# Autodesk Inventor assembly: Manipulator
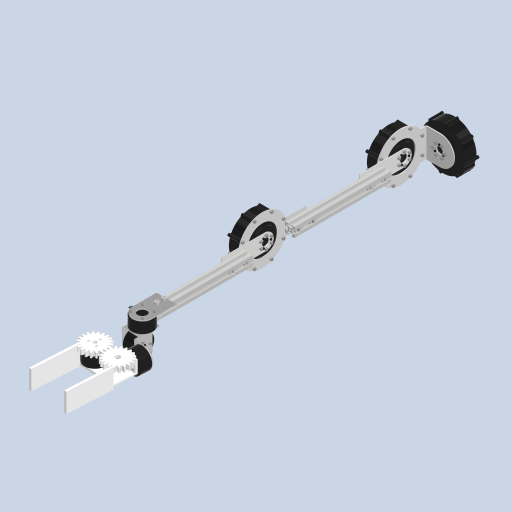
[picture p0: Inventor's stored thumbnail of the model, 512x512]
Saved by Autodesk Inventor 2023 (Build 270158000, 158)
## iProperties
Created: 2024-11-08
Part Number: Manipulator
Document SubType Name: Assembly
Designer: kiyo
Author: kiyo
## Documents named in this file (20)
- D:\GitHub\inventor\syu-si\OfficeRobot\Manipulator\Manipulator.iam
- D:\GitHub\inventor\syu-si\OfficeRobot\ReadyMade\Steadywin\GIM8108-8.iam
- D:\GitHub\inventor\syu-si\OfficeRobot\Manipulator\sholder-roll-bracket.ipt
- D:\GitHub\inventor\syu-si\OfficeRobot\Manipulator\shoulder_pitch_plate.ipt
- D:\GitHub\inventor\syu-si\OfficeRobot\Manipulator\elbow-pitch-bracket.ipt
- D:\GitHub\inventor\syu-si\OfficeRobot\Manipulator\Hand.iam
- D:\GitHub\inventor\syu-si\OfficeRobot\Manipulator\wrist-pitch-plate.ipt
- D:\GitHub\inventor\syu-si\OfficeRobot\Manipulator\wrist-yaw-plate.ipt
- D:\GitHub\inventor\syu-si\OfficeRobot\ReadyMade\Steadywin\GIM3505-8.ipt
- D:\GitHub\inventor\syu-si\OfficeRobot\Manipulator\wrist_roll_plate.ipt
- D:\GitHub\inventor\syu-si\OfficeRobot\Manipulator\HFS5-2020-200-Z5-XA10-XB40-XC160-XD190.ipt
- D:\GitHub\inventor\syu-si\OfficeRobot\ReadyMade\Screw\M3_7mm.ipt
- D:\GitHub\inventor\syu-si\OfficeRobot\ReadyMade\Screw\M3_6mm.ipt
- D:\GitHub\inventor\syu-si\OfficeRobot\ReadyMade\Screw\M2-5_4mm.ipt
- D:\GitHub\inventor\syu-si\OfficeRobot\ReadyMade\Screw\M2-5_5mm.ipt
- D:\GitHub\inventor\syu-si\OfficeRobot\ReadyMade\Screw\M2-5_7mm.ipt
- D:\GitHub\inventor\syu-si\OfficeRobot\ReadyMade\Screw\SCB5-22.ipt
- D:\GitHub\inventor\syu-si\OfficeRobot\ReadyMade\Screw\HNTP5-5.ipt
- D:\GitHub\inventor\syu-si\OfficeRobot\ReadyMade\Screw\HNTT5-5.ipt
- D:\GitHub\inventor\syu-si\OfficeRobot\ReadyMade\Screw\SCB5-8.ipt
## Components (95 placed, 19 different names)
1. GIM8108-8:1 [sub-assembly] — 挿入:1
2. GIM8108-8:2 [sub-assembly] — 挿入:2, 挿入:3, 挿入:4
3. GIM8108-8:3 [sub-assembly] — 挿入:7, 挿入:21, 挿入:22
4. sholder-roll-bracket:1 — 挿入:1, 挿入:2, 挿入:3, 肩ヨー, 挿入:94, 挿入:95, 挿入:96, 挿入:97, 挿入:98, 挿入:99, 挿入:100, 挿入:101, 挿入:102, 挿入:103, 挿入:104, 挿入:105, 挿入:106, 挿入:107
5. shoulder_pitch_plate:1 — 挿入:4, 肩ピッチ, 挿入:17, 挿入:18, 挿入:108, 挿入:109, 挿入:110, 挿入:111, 挿入:112, 挿入:113, 挿入:151, 挿入:152
6. elbow-pitch-bracket:1 — 挿入:19, 挿入:20, 挿入:21, 挿入:22, 挿入:86, 挿入:87, 挿入:88, 挿入:89, 挿入:90, 挿入:91, 挿入:92, 挿入:93, 挿入:153, 挿入:154
7. shoulder_pitch_plate:2 — 挿入:7, 肘ピッチ, 挿入:23, 挿入:24, 挿入:114, 挿入:115, 挿入:116, 挿入:117, 挿入:118, 挿入:119, 挿入:149, 挿入:150
8. GIM3505-8:1 — 挿入:63, 挿入:64, 挿入:79
9. GIM3505-8:2 — 挿入:13, 挿入:80, 挿入:81
10. GIM3505-8:3 — 挿入:16, 挿入:57, 挿入:58
11. wrist-yaw-plate:1 — メイト:1, メイト:2, フラッシュ:1, 挿入:63, 挿入:64, 挿入:120, 挿入:121, 挿入:122, 挿入:123, 挿入:161, 挿入:162, 挿入:163, 挿入:164
12. wrist_roll_plate:1 — 挿入:13, 手首ピッチ, 挿入:57, 挿入:58, 挿入:135, 挿入:136, 挿入:137, 挿入:145, 挿入:146, 挿入:147, 挿入:148
13. wrist-pitch-plate:1 — 挿入:79, 挿入:80, 挿入:81, 挿入:124, 挿入:125, 挿入:126, 挿入:127, 挿入:132, 挿入:133, 挿入:134
14. HFS5-2020-200-Z5-XA10-XB40-XC160-XD190:1 — 挿入:17, 挿入:18, 挿入:19, 挿入:20, 挿入:155, 挿入:156, 挿入:159, 挿入:160, 角度:11, 角度:12, 角度:13, 角度:14
15. HFS5-2020-200-Z5-XA10-XB40-XC160-XD190:2 — 挿入:23, 挿入:24, メイト:1, メイト:2, フラッシュ:1, 挿入:157, 挿入:158, 角度:7, 角度:8, 角度:9, 角度:10
16. Hand:1 [sub-assembly] — 挿入:16, ハンド, 挿入:128, 挿入:129, 挿入:130, 挿入:131, 挿入:138, 挿入:139, 挿入:140, 挿入:141, 挿入:142, 挿入:143, 挿入:144
17. M3_6mm:1 — 挿入:108
18. M3_6mm:2 — 挿入:110
19. M3_6mm:3 — 挿入:111
20. M3_6mm:4 — 挿入:112
21. M3_6mm:5 — 挿入:113
22. M3_6mm:6 — 挿入:109
23. M3_6mm:7 — 挿入:118
24. M3_6mm:8 — 挿入:117
25. M3_6mm:9 — 挿入:116
26. M3_6mm:10 — 挿入:115
27. M3_6mm:11 — 挿入:114
28. M3_6mm:12 — 挿入:119
29. M3_6mm:13 — 挿入:107
30. M3_6mm:14 — 挿入:106
31. M3_6mm:15 — 挿入:105
32. M3_6mm:16 — 挿入:102
33. M3_6mm:17 — 挿入:103
34. M3_6mm:18 — 挿入:104
35. M3_7mm:1 — 挿入:144
36. M3_7mm:2 — 挿入:101
37. M3_7mm:3 — 挿入:100
38. M3_7mm:4 — 挿入:99
39. M3_7mm:5 — 挿入:97
40. M3_7mm:6 — 挿入:98
41. M3_7mm:7 — 挿入:96
42. M3_7mm:8 — 挿入:95
43. M3_7mm:9 — 挿入:94
44. M3_7mm:10 — 挿入:92
45. M3_7mm:11 — 挿入:93
46. M3_7mm:12 — 挿入:86
47. M3_7mm:13 — 挿入:87
48. M3_7mm:14 — 挿入:91
49. M3_7mm:15 — 挿入:90
50. M3_7mm:16 — 挿入:89
51. M3_7mm:17 — 挿入:88
52. M2-5_4mm:21 — 挿入:147
53. M2-5_4mm:22 — 挿入:146
54. M2-5_4mm:23 — 挿入:145
55. M2-5_4mm:24 — 挿入:148
56. M2-5_4mm:1 — 挿入:120
57. M2-5_4mm:2 — 挿入:126
58. M2-5_4mm:3 — 挿入:125
59. M2-5_4mm:4 — 挿入:122
60. M2-5_4mm:5 — 挿入:121
61. M2-5_4mm:6 — 挿入:127
62. M2-5_4mm:7 — 挿入:124
63. M2-5_4mm:8 — 挿入:123
64. M2-5_4mm:9 — 挿入:129
65. M2-5_4mm:10 — 挿入:130
66. M2-5_4mm:11 — 挿入:131
67. M2-5_4mm:12 — 挿入:128
68. M2-5_5mm:1 — 挿入:132
69. M2-5_5mm:2 — 挿入:134
70. M2-5_5mm:3 — 挿入:133
71. M2-5_5mm:4 — 挿入:135
72. M2-5_5mm:5 — 挿入:137
73. M2-5_5mm:6 — 挿入:136
74. M2-5_5mm:7 — 挿入:138
75. M2-5_5mm:8 — 挿入:139
76. M2-5_5mm:9 — 挿入:140
77. M2-5_7mm:1 — 挿入:141
78. M2-5_7mm:2 — 挿入:142
79. M2-5_7mm:3 — 挿入:143
80. SCB5-22:1 — 挿入:153
81. SCB5-22:2 — 挿入:154
82. SCB5-22:3 — 挿入:152
83. SCB5-22:4 — 挿入:151
84. SCB5-22:5 — 挿入:150
85. SCB5-22:6 — 挿入:149
86. HNTP5-5:1 — 挿入:158, 角度:10
87. HNTP5-5:2 — 挿入:157, 角度:9
88. HNTP5-5:3 — 挿入:156, 角度:12
89. HNTP5-5:4 — 挿入:155, 角度:11
90. HNTP5-5:7 — 挿入:159, 角度:13
91. HNTP5-5:8 — 挿入:160, 角度:14
92. HNTT5-5:1 — 挿入:161, 角度:7
93. HNTT5-5:2 — 挿入:162, 角度:8
94. SCB5-8:1 — 挿入:163
95. SCB5-8:2 — 挿入:164
## Relationships (117: Insert 101, Angle 13, Mate 2, Flush 1)
- 挿入:1 [Insert]: GIM8108-8:1 ↔ sholder-roll-bracket:1
- 挿入:2 [Insert]: GIM8108-8:2 ↔ sholder-roll-bracket:1
- 挿入:3 [Insert]: GIM8108-8:2 ↔ sholder-roll-bracket:1
- 挿入:4 [Insert]: GIM8108-8:2 ↔ shoulder_pitch_plate:1
- 挿入:7 [Insert]: GIM8108-8:3 ↔ shoulder_pitch_plate:2
- 挿入:13 [Insert]: GIM3505-8:2 ↔ wrist_roll_plate:1
- 挿入:16 [Insert]: GIM3505-8:3 ↔ Hand:1
- 肩ヨー [Angle] (0 deg): sholder-roll-bracket:1
- 肩ピッチ [Angle] (0 deg): shoulder_pitch_plate:1
- 肘ピッチ [Angle] (0 deg): shoulder_pitch_plate:2
- 手首ピッチ [Angle] (0 deg): wrist_roll_plate:1
- ハンド [Angle] (0 deg): Hand:1
- 挿入:17 [Insert] (6 mm): shoulder_pitch_plate:1 ↔ HFS5-2020-200-Z5-XA10-XB40-XC160-XD190:1
- 挿入:18 [Insert] (6 mm): shoulder_pitch_plate:1 ↔ HFS5-2020-200-Z5-XA10-XB40-XC160-XD190:1
- 挿入:19 [Insert] (6 mm): elbow-pitch-bracket:1 ↔ HFS5-2020-200-Z5-XA10-XB40-XC160-XD190:1
- 挿入:20 [Insert] (6 mm): elbow-pitch-bracket:1 ↔ HFS5-2020-200-Z5-XA10-XB40-XC160-XD190:1
- 挿入:21 [Insert]: GIM8108-8:3 ↔ elbow-pitch-bracket:1
- 挿入:22 [Insert]: GIM8108-8:3 ↔ elbow-pitch-bracket:1
- 挿入:23 [Insert] (6 mm): shoulder_pitch_plate:2 ↔ HFS5-2020-200-Z5-XA10-XB40-XC160-XD190:2
- 挿入:24 [Insert] (6 mm): shoulder_pitch_plate:2 ↔ HFS5-2020-200-Z5-XA10-XB40-XC160-XD190:2
- メイト:1 [Mate] (-30 mm): wrist-yaw-plate:1 ↔ HFS5-2020-200-Z5-XA10-XB40-XC160-XD190:2
- メイト:2 [Mate]: wrist-yaw-plate:1 ↔ HFS5-2020-200-Z5-XA10-XB40-XC160-XD190:2
- フラッシュ:1 [Flush] (-10.5 mm): wrist-yaw-plate:1 ↔ HFS5-2020-200-Z5-XA10-XB40-XC160-XD190:2
- 挿入:57 [Insert]: GIM3505-8:3 ↔ wrist_roll_plate:1
- 挿入:58 [Insert]: GIM3505-8:3 ↔ wrist_roll_plate:1
- 挿入:63 [Insert]: GIM3505-8:1 ↔ wrist-yaw-plate:1
- 挿入:64 [Insert]: GIM3505-8:1 ↔ wrist-yaw-plate:1
- 挿入:79 [Insert]: GIM3505-8:1 ↔ wrist-pitch-plate:1
- 挿入:80 [Insert]: GIM3505-8:2 ↔ wrist-pitch-plate:1
- 挿入:81 [Insert]: GIM3505-8:2 ↔ wrist-pitch-plate:1
- 挿入:86 [Insert]: elbow-pitch-bracket:1 ↔ M3_7mm:12
- 挿入:87 [Insert]: elbow-pitch-bracket:1 ↔ M3_7mm:13
- 挿入:88 [Insert]: elbow-pitch-bracket:1 ↔ M3_7mm:17
- 挿入:89 [Insert]: elbow-pitch-bracket:1 ↔ M3_7mm:16
- 挿入:90 [Insert]: elbow-pitch-bracket:1 ↔ M3_7mm:15
- 挿入:91 [Insert]: elbow-pitch-bracket:1 ↔ M3_7mm:14
- 挿入:92 [Insert]: elbow-pitch-bracket:1 ↔ M3_7mm:10
- 挿入:93 [Insert]: elbow-pitch-bracket:1 ↔ M3_7mm:11
- 挿入:94 [Insert]: sholder-roll-bracket:1 ↔ M3_7mm:9
- 挿入:95 [Insert]: sholder-roll-bracket:1 ↔ M3_7mm:8
- 挿入:96 [Insert]: sholder-roll-bracket:1 ↔ M3_7mm:7
- 挿入:97 [Insert]: sholder-roll-bracket:1 ↔ M3_7mm:5
- 挿入:98 [Insert]: sholder-roll-bracket:1 ↔ M3_7mm:6
- 挿入:99 [Insert]: sholder-roll-bracket:1 ↔ M3_7mm:4
- 挿入:100 [Insert]: sholder-roll-bracket:1 ↔ M3_7mm:3
- 挿入:101 [Insert]: sholder-roll-bracket:1 ↔ M3_7mm:2
- 挿入:102 [Insert]: sholder-roll-bracket:1 ↔ M3_6mm:16
- 挿入:103 [Insert]: sholder-roll-bracket:1 ↔ M3_6mm:17
- 挿入:104 [Insert]: sholder-roll-bracket:1 ↔ M3_6mm:18
- 挿入:105 [Insert]: sholder-roll-bracket:1 ↔ M3_6mm:15
- 挿入:106 [Insert]: sholder-roll-bracket:1 ↔ M3_6mm:14
- 挿入:107 [Insert]: sholder-roll-bracket:1 ↔ M3_6mm:13
- 挿入:108 [Insert]: shoulder_pitch_plate:1 ↔ M3_6mm:1
- 挿入:109 [Insert]: shoulder_pitch_plate:1 ↔ M3_6mm:6
- 挿入:110 [Insert]: shoulder_pitch_plate:1 ↔ M3_6mm:2
- 挿入:111 [Insert]: shoulder_pitch_plate:1 ↔ M3_6mm:3
- 挿入:112 [Insert]: shoulder_pitch_plate:1 ↔ M3_6mm:4
- 挿入:113 [Insert]: shoulder_pitch_plate:1 ↔ M3_6mm:5
- 挿入:114 [Insert]: shoulder_pitch_plate:2 ↔ M3_6mm:11
- 挿入:115 [Insert]: shoulder_pitch_plate:2 ↔ M3_6mm:10
- 挿入:116 [Insert]: shoulder_pitch_plate:2 ↔ M3_6mm:9
- 挿入:117 [Insert]: shoulder_pitch_plate:2 ↔ M3_6mm:8
- 挿入:118 [Insert]: shoulder_pitch_plate:2 ↔ M3_6mm:7
- 挿入:119 [Insert]: shoulder_pitch_plate:2 ↔ M3_6mm:12
- 挿入:120 [Insert]: wrist-yaw-plate:1 ↔ M2-5_4mm:1
- 挿入:121 [Insert]: wrist-yaw-plate:1 ↔ M2-5_4mm:5
- 挿入:122 [Insert]: wrist-yaw-plate:1 ↔ M2-5_4mm:4
- 挿入:123 [Insert]: wrist-yaw-plate:1 ↔ M2-5_4mm:8
- 挿入:124 [Insert]: wrist-pitch-plate:1 ↔ M2-5_4mm:7
- 挿入:125 [Insert]: wrist-pitch-plate:1 ↔ M2-5_4mm:3
- 挿入:126 [Insert]: wrist-pitch-plate:1 ↔ M2-5_4mm:2
- 挿入:127 [Insert]: wrist-pitch-plate:1 ↔ M2-5_4mm:6
- 挿入:128 [Insert]: Hand:1 ↔ M2-5_4mm:12
- 挿入:129 [Insert]: Hand:1 ↔ M2-5_4mm:9
- 挿入:130 [Insert]: Hand:1 ↔ M2-5_4mm:10
- 挿入:131 [Insert]: Hand:1 ↔ M2-5_4mm:11
- 挿入:132 [Insert]: wrist-pitch-plate:1 ↔ M2-5_5mm:1
- 挿入:133 [Insert]: wrist-pitch-plate:1 ↔ M2-5_5mm:3
- 挿入:134 [Insert]: wrist-pitch-plate:1 ↔ M2-5_5mm:2
- 挿入:135 [Insert]: wrist_roll_plate:1 ↔ M2-5_5mm:4
- 挿入:136 [Insert]: wrist_roll_plate:1 ↔ M2-5_5mm:6
- 挿入:137 [Insert]: wrist_roll_plate:1 ↔ M2-5_5mm:5
- 挿入:138 [Insert]: Hand:1 ↔ M2-5_5mm:7
- 挿入:139 [Insert]: Hand:1 ↔ M2-5_5mm:8
- 挿入:140 [Insert]: Hand:1 ↔ M2-5_5mm:9
- 挿入:141 [Insert]: Hand:1 ↔ M2-5_7mm:1
- 挿入:142 [Insert]: Hand:1 ↔ M2-5_7mm:2
- 挿入:143 [Insert]: Hand:1 ↔ M2-5_7mm:3
- 挿入:144 [Insert]: Hand:1 ↔ M3_7mm:1
- 挿入:145 [Insert]: wrist_roll_plate:1 ↔ M2-5_4mm:23
- 挿入:146 [Insert]: wrist_roll_plate:1 ↔ M2-5_4mm:22
- 挿入:147 [Insert]: wrist_roll_plate:1 ↔ M2-5_4mm:21
- 挿入:148 [Insert]: wrist_roll_plate:1 ↔ M2-5_4mm:24
- 挿入:149 [Insert]: shoulder_pitch_plate:2 ↔ SCB5-22:6
- 挿入:150 [Insert]: shoulder_pitch_plate:2 ↔ SCB5-22:5
- 挿入:151 [Insert]: shoulder_pitch_plate:1 ↔ SCB5-22:4
- 挿入:152 [Insert]: shoulder_pitch_plate:1 ↔ SCB5-22:3
- 挿入:153 [Insert]: elbow-pitch-bracket:1 ↔ SCB5-22:1
- 挿入:154 [Insert]: elbow-pitch-bracket:1 ↔ SCB5-22:2
- 挿入:155 [Insert]: HFS5-2020-200-Z5-XA10-XB40-XC160-XD190:1 ↔ HNTP5-5:4
- 挿入:156 [Insert]: HFS5-2020-200-Z5-XA10-XB40-XC160-XD190:1 ↔ HNTP5-5:3
- 挿入:157 [Insert]: HFS5-2020-200-Z5-XA10-XB40-XC160-XD190:2 ↔ HNTP5-5:2
- 挿入:158 [Insert]: HFS5-2020-200-Z5-XA10-XB40-XC160-XD190:2 ↔ HNTP5-5:1
- 挿入:159 [Insert]: HFS5-2020-200-Z5-XA10-XB40-XC160-XD190:1 ↔ HNTP5-5:7
- 挿入:160 [Insert]: HFS5-2020-200-Z5-XA10-XB40-XC160-XD190:1 ↔ HNTP5-5:8
- 挿入:161 [Insert] (2 mm): wrist-yaw-plate:1 ↔ HNTT5-5:1
- 挿入:162 [Insert] (2 mm): wrist-yaw-plate:1 ↔ HNTT5-5:2
- 角度:7 [Angle] (0 deg): HFS5-2020-200-Z5-XA10-XB40-XC160-XD190:2 ↔ HNTT5-5:1
- 角度:8 [Angle] (0 deg): HFS5-2020-200-Z5-XA10-XB40-XC160-XD190:2 ↔ HNTT5-5:2
- 角度:9 [Angle] (0 deg): HFS5-2020-200-Z5-XA10-XB40-XC160-XD190:2 ↔ HNTP5-5:2
- 角度:10 [Angle] (0 deg): HFS5-2020-200-Z5-XA10-XB40-XC160-XD190:2 ↔ HNTP5-5:1
- 角度:11 [Angle] (0 deg): HFS5-2020-200-Z5-XA10-XB40-XC160-XD190:1 ↔ HNTP5-5:4
- 角度:12 [Angle] (0 deg): HFS5-2020-200-Z5-XA10-XB40-XC160-XD190:1 ↔ HNTP5-5:3
- 角度:13 [Angle] (0 deg): HFS5-2020-200-Z5-XA10-XB40-XC160-XD190:1 ↔ HNTP5-5:7
- 角度:14 [Angle] (0 deg): HFS5-2020-200-Z5-XA10-XB40-XC160-XD190:1 ↔ HNTP5-5:8
- 挿入:163 [Insert]: wrist-yaw-plate:1 ↔ SCB5-8:1
- 挿入:164 [Insert]: wrist-yaw-plate:1 ↔ SCB5-8:2
